# Autodesk Inventor assembly: SSR-40 DA Large P W S
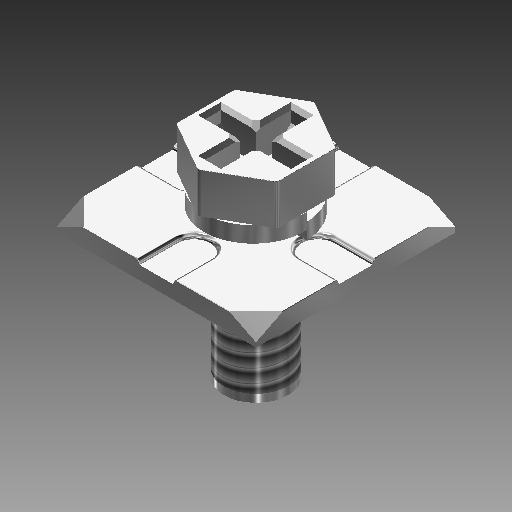
[picture p0: Inventor's stored thumbnail of the model, 512x512]
Saved by Autodesk Inventor 2019 (Build 230136000, 136)
## iProperties
Created: 2014-11-01
Part Number: SSR-40 DA Large P W S
Document SubType Name: Assembly
Designer: Tyler
Author: Tyler
## Documents named in this file (4)
- C:\Users\Ax\Google Drive\Inventor\Library\SSR-40 DA Large P W S.iam
- C:\Users\Ax\Google Drive\Inventor\Library\SSR-40 DA Screw.ipt
- C:\Users\Ax\Google Drive\Inventor\Library\SSR-40 DA Big Plate.ipt
- C:\Users\Ax\Google Drive\Inventor\Library\SSR-40 DA Lock Washer.ipt
## Components (3 placed, 3 different names)
1. SSR-40 DA Screw:1 — Mate:1, Mate:2
2. SSR-40 DA Big Plate:1 — Mate:1
3. SSR-40 DA Lock Washer:1 — Mate:2
## Relationships (2: Mate 2)
- Mate:1: SSR-40 DA Screw:1 ↔ SSR-40 DA Big Plate:1
- Mate:2: SSR-40 DA Screw:1 ↔ SSR-40 DA Lock Washer:1
